# Autodesk Inventor assembly: fan_unit_02
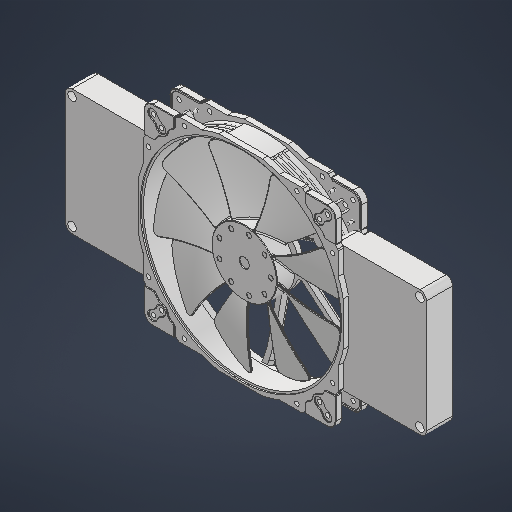
[picture p0: Inventor's stored thumbnail of the model, 512x512]
Saved by Autodesk Inventor 2026.2 (Build 302298010, 298A)
## iProperties
Created: 2026-05-14
Part Number: fan_unit_02
Document SubType Name: Assembly
Designer: nyxeon
Author: nyxeon
## Documents named in this file (3)
- C:\Users\nyxeon\Documents\CAD\Inventor\eatx_case\robocup\fan_unit_02.iam
- C:\Users\nyxeon\Documents\CAD\Inventor\eatx_case\robocup\parts\fan_noctua_nf-a20_assembly\fan_noctua_nf-a20_assembly\fan_noctua_nf-a20_assembly.iam
- C:\Users\nyxeon\Documents\CAD\Inventor\eatx_case\robocup\fan_connector_03.ipt
## Components (3 placed, 2 different names)
1. fan_noctua_nf-a20_assembly:1 [sub-assembly] — メイト:1, メイト:2, メイト:3, メイト:4, メイト:5, メイト:6
2. fan_connector_03:1 — メイト:1, メイト:3, メイト:4
3. fan_connector_03:2 — メイト:2, メイト:5, メイト:6
## Relationships (6: Mate 6)
- メイト:1 [Mate]: fan_noctua_nf-a20_assembly:1 ↔ fan_connector_03:1
- メイト:2 [Mate]: fan_noctua_nf-a20_assembly:1 ↔ fan_connector_03:2
- メイト:3 [Mate]: fan_noctua_nf-a20_assembly:1 ↔ fan_connector_03:1
- メイト:4 [Mate]: fan_noctua_nf-a20_assembly:1 ↔ fan_connector_03:1
- メイト:5 [Mate]: fan_noctua_nf-a20_assembly:1 ↔ fan_connector_03:2
- メイト:6 [Mate]: fan_noctua_nf-a20_assembly:1 ↔ fan_connector_03:2
